# Autodesk Inventor assembly: FrontMiddleShaft
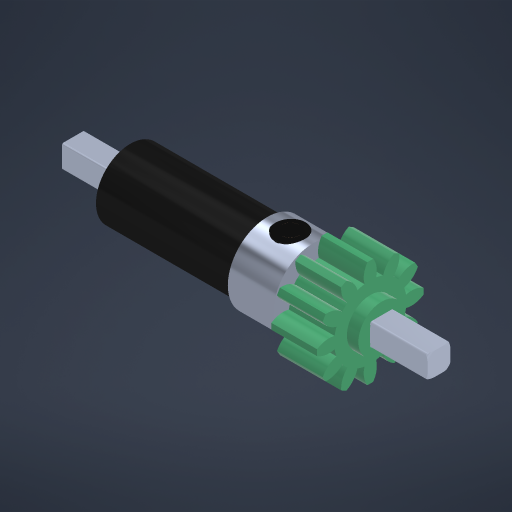
[picture p0: Inventor's stored thumbnail of the model, 512x512]
Saved by Autodesk Inventor 2023 (Build 270158000, 158)
## iProperties
Created: 2023-05-11
Part Number: FrontMiddleShaft
Document SubType Name: Assembly
Designer: alex
Author: alex
## Documents named in this file (8)
- C:\Users\alex\Documents\GitHub\4067X-Over-Under-CAD\Chassis\FrontMiddleShaft.iam
- C:\Users\alex\Documents\GitHub\4067X-Over-Under-CAD\VEX-CAD-Inventor\Motion\Gears\LS 12T Gear.ipt
- C:\Users\alex\Documents\GitHub\4067X-Over-Under-CAD\VEX-CAD-Inventor\Motion\Shaft LS\Shaft Collar ipts\Shaft Collar Set Screw.ipt
- C:\Users\alex\Documents\GitHub\4067X-Over-Under-CAD\VEX-CAD-Inventor\Motion\Spacers\Spacer Nylon .375 OD\NSpacer .375 OD x .500.ipt
- C:\Users\alex\Documents\GitHub\4067X-Over-Under-CAD\VEX-CAD-Inventor\Motion\Spacers\Spacer Nylon .375 OD.ipt
- C:\Users\alex\Documents\GitHub\4067X-Over-Under-CAD\VEX-CAD-Inventor\Motion\Spacers\Spacer Nylon .375 OD\NSpacer .375 OD x .250.ipt
- C:\Users\alex\Documents\GitHub\4067X-Over-Under-CAD\VEX-CAD-Inventor\Motion\Shaft LS\Shaft LS\Shaft LS 2.0.ipt
- C:\Users\alex\Documents\GitHub\4067X-Over-Under-CAD\VEX-CAD-Inventor\Motion\Shaft LS\Shaft LS.ipt
## Components (5 placed, 5 different names)
1. LS 12T Gear:1 — Insert:1, Mate:1, Mate:2, Flush:1
2. Shaft Collar Set Screw:1 — Insert:1, Insert:2
3. NSpacer .375 OD x .500:1 — Insert:2, Insert:3
4. NSpacer .375 OD x .250:2 — Insert:3
5. Shaft LS 2.0:1 — Mate:1, Mate:2, Flush:1
## Relationships (6: Insert 3, Mate 2, Flush 1)
- Insert:1: LS 12T Gear:1 ↔ Shaft Collar Set Screw:1
- Insert:2: Shaft Collar Set Screw:1 ↔ NSpacer .375 OD x .500:1
- Insert:3: NSpacer .375 OD x .500:1 ↔ NSpacer .375 OD x .250:2
- Mate:1: LS 12T Gear:1 ↔ Shaft LS 2.0:1
- Mate:2: LS 12T Gear:1 ↔ Shaft LS 2.0:1
- Flush:1 (-7.9375 mm): LS 12T Gear:1 ↔ Shaft LS 2.0:1
